# Autodesk Inventor assembly: TapeMeasureAssemblyVersion1
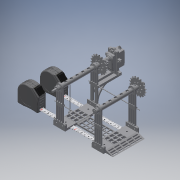
[picture p0: Inventor's stored thumbnail of the model, 180x180]
Saved by Autodesk Inventor 2019 (Build 230136000, 136)
## iProperties
Created: 2018-11-08
Part Number: TapeMeasureAssemblyVersion1
Document SubType Name: Assembly
Designer: Ashley
Author: Ashley
## Documents named in this file (18)
- C:\Users\mrhftc\repositories\design\inventor\2018-2019\Tape Measure Braket\Version Three\Tape Measure Bracket Assembly V3.iam
- C:\Users\mrhftc\repositories\design\inventor\2018-2019\Tape Measure Braket\Version Three\Bracket Bottom V3.ipt
- C:\Users\mrhftc\repositories\design\inventor\2018-2019\Tape Measure Braket\Tape Measure\Tape Measure Edited.iam
- C:\Users\mrhftc\repositories\design\inventor\2018-2019\Tape Measure Braket\Version Three\Side V3.ipt
- C:\Users\mrhftc\repositories\design\inventor\Imported Components\goBilda\Bearing6mmID.ipt
- C:\Users\mrhftc\repositories\design\inventor\2018-2019\Tape Measure Braket\Finished Parts\Spinner94mmDShaft.ipt
- C:\Users\mrhftc\repositories\design\inventor\Imported Components\goBilda\DShaft140mm.ipt
- C:\Users\mrhftc\repositories\design\inventor\Imported Components\goBilda\Collar6mm\SetScrewCollar6mmboreassembly.iam
- C:\Users\mrhftc\repositories\design\inventor\Imported Components\goBilda\DShaft160mm.ipt
- C:\Users\mrhftc\repositories\design\inventor\2018-2019\Tape Measure Braket\Finished Parts\2mmAxel.ipt
- C:\Users\mrhftc\repositories\design\inventor\Imported Components\goBilda\CampingHub\ClampingHub assembly.iam
- C:\Users\mrhftc\repositories\design\inventor\Imported Components\goBilda\8mmPlasticPitchSproket.ipt
- C:\Users\mrhftc\repositories\design\inventor\Imported Components\goBilda\Servo To Shaft\ServoToShaftCoupler.iam
- C:\Users\mrhftc\repositories\design\inventor\Imported Components\goBilda\goBildaServo.ipt
- C:\Users\mrhftc\repositories\design\inventor\Imported Components\goBilda\1802SeriesServoFrame.ipt
- C:\Users\mrhftc\repositories\design\inventor\2018-2019\Tape Measure Braket\Version Three\Side Servo V3.ipt
- C:\Users\mrhftc\repositories\design\inventor\2018-2019\Tape Measure Braket\Version Three\Braket Top V3.ipt
- C:\Users\mrhftc\repositories\design\inventor\2018-2019\Tape Measure Braket\Finished Parts\2mmAxel3in.ipt
## Components (33 placed, 30 different names)
1. Bracket Bottom — Mate:1, Mate:4, Mate:5, Insert:24
2. Tape Measure Right [sub-assembly]
3. Tape Measure Left [sub-assembly]
4. Back Right Side
5. Front Right Side — Mate:1, Insert:2, Insert:11
6. Front Left Side — Insert:3, Insert:10
7. Back Right Bearing — Insert:17
8. Front Right Bearing — Insert:2
9. Front Left Beaing — Insert:3
10. Front Left BEaring — Insert:23
11. Back Spinner — Insert:22
12. Front Spinner — Insert:6
13. Front Right Collar [sub-assembly]
14. Front Axel — Insert:6, Insert:8, Insert:14
15. Front Left Collar [sub-assembly] — Insert:8
16. Back Left Collar [sub-assembly]
17. Back Right Collar [sub-assembly] — Insert:18
18. Back Axel — Insert:17, Insert:18, Insert:19, Insert:20, Insert:22
19. Left axel — Insert:10
20. Right Axel — Insert:11
21. Front Sproket — Insert:12
22. Front Claming Hub [sub-assembly] — Insert:12, Insert:14
23. Back Sproket
24. Back Clamping Hub [sub-assembly] — Insert:19
25. Servo To Shaft Coupler [sub-assembly] — Insert:20, Insert:21
26. Servo — Insert:21, Mate:3
27. Servo Frame — Mate:3
28. Side Servo V3:1 — Insert:23
29. Braket Top V3:1 — Mate:5
30. Braket Top V3:2 — Mate:4
31. Braket Top V3:3
32. Braket Top V3:4
33. 2mmAxel3in:1 — Insert:24
## Relationships (21: Insert 17, Mate 4)
- Mate:1: Bracket Bottom ↔ Front Right Side
- Insert:2: Front Right Side ↔ Front Right Bearing
- Insert:3: Front Left Side ↔ Front Left Beaing
- Insert:6 (17 mm): Front Spinner ↔ Front Axel
- Insert:8 (14 mm): Front Axel ↔ Front Left Collar
- Insert:10 (-30 mm): Front Left Side ↔ Left axel
- Insert:11 (-30 mm): Front Right Side ↔ Right Axel
- Insert:12 (-1 mm): Front Sproket ↔ Front Claming Hub
- [Insert] (-1 mm): Back Sproket ↔ Back Clamping Hub
- Insert:14 (1 mm): Front Axel ↔ Front Claming Hub
- Insert:17 (20 mm): Back Right Bearing ↔ Back Axel
- Insert:18 (12 mm): Back Right Collar ↔ Back Axel
- Insert:19 (11 mm): Back Axel ↔ Back Clamping Hub
- Insert:20 (-6 mm): Back Axel ↔ Servo To Shaft Coupler
- Insert:21 (-3 mm): Servo To Shaft Coupler ↔ Servo
- Mate:3: Servo ↔ Servo Frame
- Insert:22 (40 mm): Back Spinner ↔ Back Axel
- Insert:23: Front Left BEaring ↔ Side Servo V3:1
- Mate:4: Bracket Bottom ↔ Braket Top V3:2
- Mate:5: Bracket Bottom ↔ Braket Top V3:1
- Insert:24 (-6.5 mm): Bracket Bottom ↔ 2mmAxel3in:1
## Named parameters: d26_d25 = -1 mm
